# Autodesk Inventor assembly: Portaherramienta com
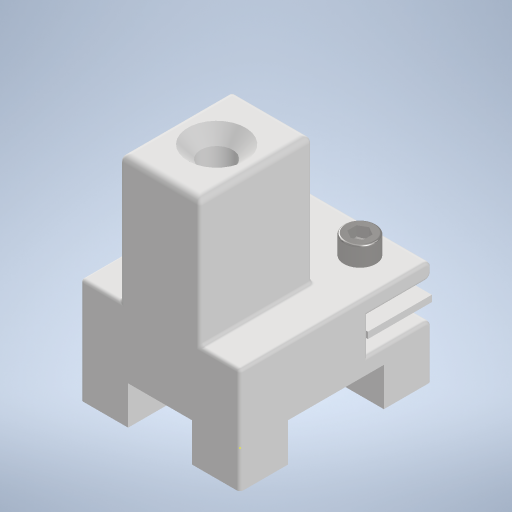
[picture p0: Inventor's stored thumbnail of the model, 512x512]
Saved by Autodesk Inventor 2024 (Build 280153000, 153)
## iProperties
Created: 2023-11-25
Part Number: Portaherramienta com
Document SubType Name: Assembly
Designer: Juan_Daleman
Author: Juan_Daleman
## Documents named in this file (4)
- D:\Documentos\Proyectos_U\Semestre 9\Robotica\Lab\Lab5\Portaherramienta com.iam
- D:\Documentos\Proyectos_U\Semestre 9\Robotica\Lab\Lab5\PortaHerramienta1.ipt
- D:\Documentos\Inventor\Content Center Files\R2024\en-US\AS 1420\AS 1420 - 1973 - M6 x 10.ipt
- D:\Documentos\Proyectos_U\Semestre 9\Robotica\Lab\Lab5\PortaHerramienta2.ipt
## Components (4 placed, 3 different names)
1. PortaHerramienta1:1 — Insert:1, Insert:2, Mate:1, Mate:2, Flush:1
2. AS 1420 - Metric M6 x 10:1 — Insert:1
3. AS 1420 - Metric M6 x 10:2 — Insert:2
4. PortaHerramienta2:1 — Mate:1, Mate:2, Flush:1
## Relationships (5: Insert 2, Mate 2, Flush 1)
- Insert:1: PortaHerramienta1:1 ↔ AS 1420 - Metric M6 x 10:1
- Insert:2: PortaHerramienta1:1 ↔ AS 1420 - Metric M6 x 10:2
- Mate:1 (4.5 mm): PortaHerramienta1:1 ↔ PortaHerramienta2:1
- Mate:2: PortaHerramienta1:1 ↔ PortaHerramienta2:1
- Flush:1: PortaHerramienta1:1 ↔ PortaHerramienta2:1
